# Autodesk Inventor assembly: cadena conjunto
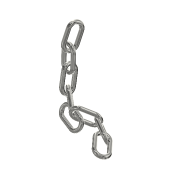
[picture p0: Inventor's stored thumbnail of the model, 180x180]
Saved by Autodesk Inventor 2016 (Build 200138000, 138)
## iProperties
Created: 2015-11-26
Part Number: cadena conjunto
Document SubType Name: Assembly
Designer: H. Valenzuela B.
Author: H. Valenzuela B.
## Documents named in this file (2)
- Z:\DIBUJOS\912_Clientes\C11_Geotec\87_Mesa Saca testigo Nueva\Mesa saca testigo 4\Mesa Hidraulica Saca Testigo - copia\Modelos\cadena.iam
- Z:\DIBUJOS\912_Clientes\C11_Geotec\87_Mesa Saca testigo Nueva\Mesa saca testigo 4\Mesa Hidraulica Saca Testigo - copia\Modelos\cadena.ipt
## Components (8 placed, 1 different names)
1. cadena:5
2. cadena:8
3. cadena:9
4. cadena:13
5. cadena:15
6. cadena:16
7. cadena:17
8. cadena:18
## Relationships (4: Tangent 4)
- [Tangent]: cadena:8 ↔ cadena:9
- [Tangent]: cadena:15 ↔ cadena:16
- [Tangent]: cadena:17 ↔ cadena:18
- [Tangent]: cadena:16 ↔ cadena:17
## Named parameters: d8_d2 = 0 mm, d12_d6_d3_d2 = 0 mm, d13_d7_d4 = 0 mm, d14_d8_d2 = 0 mm
